# Autodesk Inventor assembly: A1-19027-100-00 Spool SP-237-2-P-126-1-B
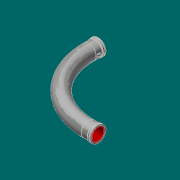
[picture p0: Inventor's stored thumbnail of the model, 180x180]
Saved by Autodesk Inventor 2017.3 (Build 213257000, 257)
## iProperties
Created: 2019-10-16
Part Number: A1-19027-100-00 Spool SP-237-2-P-126-1-B
Document SubType Name: Weldment
Designer: GVD
Weld Material: Steel, Mild, Welded
Mass: 9.33142e+06 g
Surface Area: 827233 cm^2
Volume: 1.24978e+06 cm^3
Density: 7.46643 g/cm^3
Author: GVD
## Documents named in this file (12)
- N:\A1 - Projects\A1-19\A1-19027--Syncrude Aurora HT2 spools - SP-237\A1-19027-100-00 Spool SP-237-2-P-126-1-B.iam
- N:\A1 - Projects\A1-19\A1-19027--Syncrude Aurora HT2 spools - SP-237\A1-19027-100-01 36in elbow.ipt
- N:\A1 - Projects\A1-19\A1-19027--Syncrude Aurora HT2 spools - SP-237\A1-19027-100-02 36in pipe.ipt
- N:\A1 - Projects\A1-19\A1-19027--Syncrude Aurora HT2 spools - SP-237\A1-19027-100-03 36in Type B victaulic ring.ipt
- N:\A1 - Projects\A1-19\A1-19027--Syncrude Aurora HT2 spools - SP-237\A1-19027-100-04 HCWI elbow - male.ipt
- N:\A1 - Projects\A1-19\A1-19027--Syncrude Aurora HT2 spools - SP-237\A1-19027-100-05 HCWI elbow - female.ipt
- N:\A1 - Projects\A1-19\A1-19027--Syncrude Aurora HT2 spools - SP-237\A1-19027-100-06 HCWI liner - pup.ipt
- N:\A1 - Projects\A1-19\A1-19027--Syncrude Aurora HT2 spools - SP-237\A1-19027-100-07 2in x 36in threadolet.ipt
- N:\Inventor\Content Center Files\R2017\en-US\ASME B16.11(23)\ASME B16.11 Hex Head Plug 2.ipt
- N:\Inventor\Content Center Files\R2017\en-US\ASME B16.11(23)\ASME B16.11 Hex Head Plug 3_4.ipt
- N:\Penticton Foundry\Tag mount - 6in.ipt
- N:\A1 - Projects\A1-19\A1-19027--Syncrude Aurora HT2 spools - SP-237\A1-19027-100-08 HCWI elbow - center.ipt
## Components (34 placed, 11 different names)
1. A1-19027-100-01 36in elbow:1 — Insert:1, Angle:1, Insert:2, Angle:2, Angle:3, Angle:4, Flush:1, Mate:1, Angle:5, Flush:2, Flush:3, Mate:2, Mate:3, Mate:4, Angle:9, Mate:5, Angle:11, Angle:12, Mate:6, Angle:13, Mate:7, Tangent:3, Mate:8, Tangent:4, Mate:9, Mate:10, Tangent:5, Tangent:6
2. A1-19027-100-02 36in pipe:1 — Insert:1, Angle:1, Insert:3, Tangent:1, Flush:5, Tangent:2
3. A1-19027-100-02 36in pipe:2 — Insert:2, Angle:2, Insert:4
4. A1-19027-100-03 36in Type B victaulic ring:1 — Insert:3, Angle:3, Flush:6
5. A1-19027-100-03 36in Type B victaulic ring:2 — Insert:4, Angle:4
6. A1-19027-100-04 HCWI elbow - male:1 — Flush:1, Mate:1, Angle:5, Angle:6, Insert:6, Angle:7, Angle:8, Flush:7, Mate:11, Insert:9
7. A1-19027-100-08 HCWI elbow - center:1 — Flush:7, Mate:11, Insert:9, Insert:10
8. A1-19027-100-05 HCWI elbow - female:1 — Angle:6, Insert:7, Insert:10
9. A1-19027-100-06 HCWI liner - pup:1 — Insert:6, Angle:7
10. A1-19027-100-06 HCWI liner - pup:2 — Insert:7, Angle:8
11. A1-19027-100-07 2in x 36in threadolet:1 — Mate:3, Mate:4, Angle:9, Insert:8, Angle:10
12. ASME B16.11 Hex Head Plug 2:1 — Insert:8, Angle:10
13. ASME B16.11 Hex Head Plug 3/4:11 — Mate:7, Angle:14, Tangent:3
14. ASME B16.11 Hex Head Plug 3/4:13 — Mate:8, Angle:15, Tangent:4
15. ASME B16.11 Hex Head Plug 3/4:14 — Mate:10, Tangent:5, Angle:16
16. ASME B16.11 Hex Head Plug 3/4:15 — Mate:9, Tangent:6, Angle:17
17. Tag mount - 6in:1 — Flush:5, Flush:6, Tangent:2
18. Tag mount - 6in:2
19. ASME B16.11 Hex Head Plug 3/4:2 — Mate:6, Flush:4, Angle:13
20. ASME B16.11 Hex Head Plug 3/4:5
21. ASME B16.11 Hex Head Plug 3/4:9
22. ASME B16.11 Hex Head Plug 3/4:10
23. ASME B16.11 Hex Head Plug 3/4:1 — Mate:5, Angle:11, Tangent:1, Angle:12, Flush:4
24. ASME B16.11 Hex Head Plug 3/4:3
25. ASME B16.11 Hex Head Plug 3/4:4
26. ASME B16.11 Hex Head Plug 3/4:6
27. ASME B16.11 Hex Head Plug 3/4:7
28. ASME B16.11 Hex Head Plug 3/4:8
29. ASME B16.11 Hex Head Plug 3/4:16
30. ASME B16.11 Hex Head Plug 3/4:17
31. ASME B16.11 Hex Head Plug 3/4:18
32. ASME B16.11 Hex Head Plug 3/4:19
33. ASME B16.11 Hex Head Plug 3/4:20
34. ASME B16.11 Hex Head Plug 3/4:21
## Component patterns: (2 elements, first: Tag mount - 6in:1), (2 elements), (2 elements), (2 elements, first: ASME B16.11 Hex Head Plug 3/4:2), Component Pattern 2:2 (2 elements), (2 elements), Component Pattern 6:2 (2 elements), (3 elements, first: ASME B16.11 Hex Head Plug 3/4:1), Component Pattern 1:2 (3 elements), Component Pattern 1:3 (3 elements), Component Pattern 1:4 (3 elements)
## Relationships (50: Angle 17, Mate 11, Insert 9, Flush 7, Tangent 6)
- Insert:1 (2.3813 mm): A1-19027-100-01 36in elbow:1 ↔ A1-19027-100-02 36in pipe:1
- Angle:1 (0 deg): A1-19027-100-01 36in elbow:1 ↔ A1-19027-100-02 36in pipe:1
- Insert:2 (2.3813 mm): A1-19027-100-01 36in elbow:1 ↔ A1-19027-100-02 36in pipe:2
- Angle:2 (0 deg): A1-19027-100-01 36in elbow:1 ↔ A1-19027-100-02 36in pipe:2
- Insert:3 (2.3813 mm): A1-19027-100-02 36in pipe:1 ↔ A1-19027-100-03 36in Type B victaulic ring:1
- Angle:3 (0 deg): A1-19027-100-01 36in elbow:1 ↔ A1-19027-100-03 36in Type B victaulic ring:1
- Insert:4 (2.3813 mm): A1-19027-100-02 36in pipe:2 ↔ A1-19027-100-03 36in Type B victaulic ring:2
- Angle:4 (0 deg): A1-19027-100-01 36in elbow:1 ↔ A1-19027-100-03 36in Type B victaulic ring:2
- Flush:1: A1-19027-100-01 36in elbow:1 ↔ A1-19027-100-04 HCWI elbow - male:1
- Mate:1: A1-19027-100-01 36in elbow:1 ↔ A1-19027-100-04 HCWI elbow - male:1
- Angle:5 (0 deg): A1-19027-100-01 36in elbow:1 ↔ A1-19027-100-04 HCWI elbow - male:1
- Angle:6 (180 deg): A1-19027-100-04 HCWI elbow - male:1 ↔ A1-19027-100-05 HCWI elbow - female:1
- Insert:6: A1-19027-100-04 HCWI elbow - male:1 ↔ A1-19027-100-06 HCWI liner - pup:1
- Angle:7 (0 deg): A1-19027-100-04 HCWI elbow - male:1 ↔ A1-19027-100-06 HCWI liner - pup:1
- Insert:7: A1-19027-100-05 HCWI elbow - female:1 ↔ A1-19027-100-06 HCWI liner - pup:2
- Angle:8 (0 deg): A1-19027-100-04 HCWI elbow - male:1 ↔ A1-19027-100-06 HCWI liner - pup:2
- Flush:2: A1-19027-100-01 36in elbow:1
- Flush:3: A1-19027-100-01 36in elbow:1
- Mate:2: A1-19027-100-01 36in elbow:1
- Mate:3: A1-19027-100-01 36in elbow:1 ↔ A1-19027-100-07 2in x 36in threadolet:1
- Mate:4: A1-19027-100-01 36in elbow:1 ↔ A1-19027-100-07 2in x 36in threadolet:1
- Angle:9 (0 deg): A1-19027-100-01 36in elbow:1 ↔ A1-19027-100-07 2in x 36in threadolet:1
- Insert:8 (-15.494 mm): A1-19027-100-07 2in x 36in threadolet:1 ↔ ASME B16.11 Hex Head Plug 2:1
- Angle:10 (0 deg): A1-19027-100-07 2in x 36in threadolet:1 ↔ ASME B16.11 Hex Head Plug 2:1
- Mate:5: A1-19027-100-01 36in elbow:1 ↔ ASME B16.11 Hex Head Plug 3/4:1
- Angle:11 (180 deg): A1-19027-100-01 36in elbow:1 ↔ ASME B16.11 Hex Head Plug 3/4:1
- Tangent:1 (-12.2428 mm): A1-19027-100-02 36in pipe:1 ↔ ASME B16.11 Hex Head Plug 3/4:1
- Angle:12 (0 deg): A1-19027-100-01 36in elbow:1 ↔ ASME B16.11 Hex Head Plug 3/4:1
- Mate:6: A1-19027-100-01 36in elbow:1 ↔ ASME B16.11 Hex Head Plug 3/4:2
- Flush:4: ASME B16.11 Hex Head Plug 3/4:2 ↔ ASME B16.11 Hex Head Plug 3/4:1
- Angle:13 (0 deg): A1-19027-100-01 36in elbow:1 ↔ ASME B16.11 Hex Head Plug 3/4:2
- Flush:5: A1-19027-100-02 36in pipe:1 ↔ Tag mount - 6in:1
- Flush:6 (355.6 mm): A1-19027-100-03 36in Type B victaulic ring:1 ↔ Tag mount - 6in:1
- Tangent:2: A1-19027-100-02 36in pipe:1 ↔ Tag mount - 6in:1
- Mate:7: A1-19027-100-01 36in elbow:1 ↔ ASME B16.11 Hex Head Plug 3/4:11
- Angle:14 (45 deg): ASME B16.11 Hex Head Plug 3/4:11
- Tangent:3: A1-19027-100-01 36in elbow:1 ↔ ASME B16.11 Hex Head Plug 3/4:11
- Mate:8: A1-19027-100-01 36in elbow:1 ↔ ASME B16.11 Hex Head Plug 3/4:13
- Angle:15 (135 deg): ASME B16.11 Hex Head Plug 3/4:13
- Tangent:4: A1-19027-100-01 36in elbow:1 ↔ ASME B16.11 Hex Head Plug 3/4:13
- Mate:9: A1-19027-100-01 36in elbow:1 ↔ ASME B16.11 Hex Head Plug 3/4:15
- Mate:10: A1-19027-100-01 36in elbow:1 ↔ ASME B16.11 Hex Head Plug 3/4:14
- Tangent:5: A1-19027-100-01 36in elbow:1 ↔ ASME B16.11 Hex Head Plug 3/4:14
- Angle:16 (45 deg): ASME B16.11 Hex Head Plug 3/4:14
- Tangent:6: A1-19027-100-01 36in elbow:1 ↔ ASME B16.11 Hex Head Plug 3/4:15
- Angle:17 (135 deg): ASME B16.11 Hex Head Plug 3/4:15
- Flush:7: A1-19027-100-04 HCWI elbow - male:1 ↔ A1-19027-100-08 HCWI elbow - center:1
- Mate:11: A1-19027-100-04 HCWI elbow - male:1 ↔ A1-19027-100-08 HCWI elbow - center:1
- Insert:9: A1-19027-100-04 HCWI elbow - male:1 ↔ A1-19027-100-08 HCWI elbow - center:1
- Insert:10: A1-19027-100-08 HCWI elbow - center:1 ↔ A1-19027-100-05 HCWI elbow - female:1
